# Autodesk Inventor assembly: Kreiselpumpe
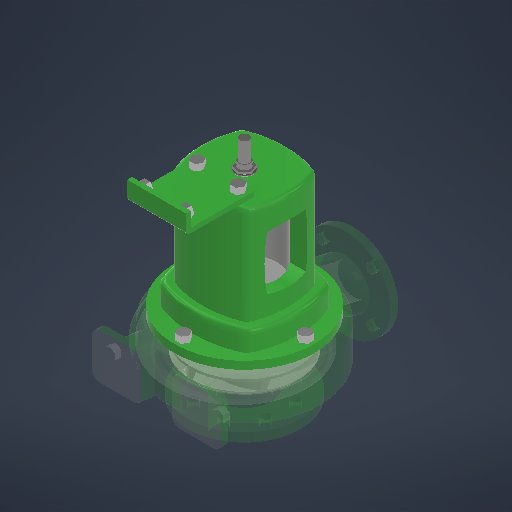
[picture p0: Inventor's stored thumbnail of the model, 512x512]
Saved by Autodesk Inventor 2026 (Build 300175050, 175E)
## iProperties
Created: 2025-11-20
Part Number: Kreiselpumpe
Document SubType Name: Assembly
Designer: aurich
Author: aurich
## Documents named in this file (7)
- D:\Unity Projekte\Pipemaster\Assets\Modelle\Kreiselpumpe AR\Geometry\Kreiselpumpe.iam
- D:\Unity Projekte\Pipemaster\Assets\Modelle\Kreiselpumpe AR\Geometry\Spiralgehause.ipt
- D:\Unity Projekte\Pipemaster\Assets\Modelle\Kreiselpumpe AR\Geometry\Lagerung.ipt
- D:\Unity Projekte\Pipemaster\Assets\Modelle\Kreiselpumpe AR\Geometry\Laufrad_Deckscheibe_hinten.ipt
- D:\Unity Projekte\Pipemaster\Assets\Modelle\Kreiselpumpe AR\Geometry\Laufrad_Deckscheibe_vorne.ipt
- D:\Unity Projekte\Pipemaster\Assets\Modelle\Kreiselpumpe AR\Geometry\Laufrad_Schaufeln.ipt
- D:\Unity Projekte\Pipemaster\Assets\Modelle\Kreiselpumpe AR\Geometry\Welle.ipt
## Components (6 placed, 6 different names)
1. Spiralgehause:1 — Passend:1, Passend:2, Fluchtend:1, Passend:5, Passend:6, Fluchtend:7
2. Lagerung:1 — Passend:1, Passend:2, Fluchtend:1
3. Laufrad_Deckscheibe_hinten:1 — Passend:3, Passend:4, Fluchtend:2, Fluchtend:4, Fluchtend:5, Passend:5, Fluchtend:6, Passend:7
4. Laufrad_Deckscheibe_vorne:1 — Passend:3, Fluchtend:2, Fluchtend:3, Fluchtend:4, Passend:6, Passend:9
5. Laufrad_Schaufeln:1 — Passend:4, Fluchtend:3, Fluchtend:5
6. Welle:1 — Fluchtend:6, Passend:7, Passend:8
## Relationships (16: Mate 9, Flush 7)
- Passend:1 [Mate]: Spiralgehause:1 ↔ Lagerung:1
- Passend:2 [Mate]: Spiralgehause:1 ↔ Lagerung:1
- Fluchtend:1 [Flush]: Spiralgehause:1 ↔ Lagerung:1
- Passend:3 [Mate]: Laufrad_Deckscheibe_hinten:1 ↔ Laufrad_Deckscheibe_vorne:1
- Passend:4 [Mate]: Laufrad_Deckscheibe_hinten:1 ↔ Laufrad_Schaufeln:1
- Fluchtend:2 [Flush]: Laufrad_Deckscheibe_hinten:1 ↔ Laufrad_Deckscheibe_vorne:1
- Fluchtend:3 [Flush]: Laufrad_Deckscheibe_vorne:1 ↔ Laufrad_Schaufeln:1
- Fluchtend:4 [Flush]: Laufrad_Deckscheibe_hinten:1 ↔ Laufrad_Deckscheibe_vorne:1
- Fluchtend:5 [Flush]: Laufrad_Deckscheibe_hinten:1 ↔ Laufrad_Schaufeln:1
- Passend:5 [Mate]: Spiralgehause:1 ↔ Laufrad_Deckscheibe_hinten:1
- Passend:6 [Mate] (1 mm): Spiralgehause:1 ↔ Laufrad_Deckscheibe_vorne:1
- Fluchtend:6 [Flush]: Laufrad_Deckscheibe_hinten:1 ↔ Welle:1
- Passend:7 [Mate]: Laufrad_Deckscheibe_hinten:1 ↔ Welle:1
- Passend:8 [Mate]: Welle:1
- Passend:9 [Mate]: Laufrad_Deckscheibe_vorne:1
- Fluchtend:7 [Flush]: Spiralgehause:1
